# Autodesk Inventor assembly: bottom_shell
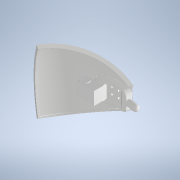
[picture p0: Inventor's stored thumbnail of the model, 180x180]
Saved by Autodesk Inventor 2020.2 (Build 242310000, 310)
## iProperties
Created: 2020-11-22
Part Number: bottom_shell
Document SubType Name: Assembly
Designer: mazzo
Author: mazzo
## Documents named in this file (4)
- D:\Documenti\università\Progetto Meccanica dei Robot\assembled in urdf\bottom_shell.iam
- D:\Documenti\università\Progetto Meccanica dei Robot\meccanica\parti autodesk\V6\V6 Luca\bottom_shell.ipt
- D:\Documenti\università\Progetto Meccanica dei Robot\meccanica\parti autodesk\V6\V6 Luca\end_effector.ipt
- D:\Documenti\università\Progetto Meccanica dei Robot\meccanica\parti autodesk\V6\V6 Luca\Motore1.ipt
## Components (3 placed, 3 different names)
1. bottom_shell:1 — Coincidente:5, Coincidente:6, Coincidente:7
2. end_effector:1 — Coincidente:2, Coincidente:3, Coincidente:4, Coincidente:5, Coincidente:6, Coincidente:7
3. Motore1:1 — Coincidente:1, Allineato:1, Angolo:1, Coincidente:2, Coincidente:3, Coincidente:4
## Relationships (9: Mate 7, Flush 1, Angle 1)
- Coincidente:1 [Mate]: Motore1:1
- Allineato:1 [Flush]: Motore1:1
- Angolo:1 [Angle] (180 deg): Motore1:1
- Coincidente:2 [Mate]: end_effector:1 ↔ Motore1:1
- Coincidente:3 [Mate]: end_effector:1 ↔ Motore1:1
- Coincidente:4 [Mate]: end_effector:1 ↔ Motore1:1
- Coincidente:5 [Mate]: bottom_shell:1 ↔ end_effector:1
- Coincidente:6 [Mate]: bottom_shell:1 ↔ end_effector:1
- Coincidente:7 [Mate]: bottom_shell:1 ↔ end_effector:1
